# Autodesk Inventor assembly: prowadzenie
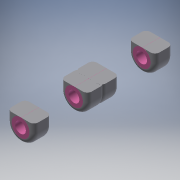
[picture p0: Inventor's stored thumbnail of the model, 180x180]
Saved by Autodesk Inventor 2019 (Build 230136000, 136)
## iProperties
Created: 2020-01-12
Part Number: prowadzenie
Material: Ogólny
Document SubType Name: Assembly
Designer: Karolina
Author: Karolina
## Documents named in this file (3)
- C:\Users\Karolina\Desktop\Kuba\rekav2\dlon\prowadzenie.iam
- C:\Users\Karolina\Desktop\Kuba\rekav2\dlon\lozysko.ipt
- C:\Users\Karolina\Desktop\Kuba\rekav2\dlon\trzym.ipt
## Components (8 placed, 2 different names)
1. trzym:1 — Równoległy:3, Zestawiający:3, Zestawiający:5, Zestawiający:8, Równoległy:5
2. trzym:2 — Równoległy:2, Zestawiający:3, Zestawiający:4, Zestawiający:6, Zestawiający:7, Równoległy:7
3. trzym:3 — Zestawiający:1, Zestawiający:2, Równoległy:1, Równoległy:2, Zestawiający:6, Zestawiający:9, Zestawiający:10, Równoległy:4
4. trzym:4 — Zestawiający:1, Zestawiający:2, Równoległy:1, Równoległy:3, Zestawiający:4, Zestawiający:5, Równoległy:6
5. lozysko:1 — Zestawiający:10, Równoległy:4
6. lozysko:2 — Zestawiający:9, Równoległy:6
7. lozysko:3 — Zestawiający:8, Równoległy:7
8. lozysko:4 — Zestawiający:7, Równoległy:5
## Relationships (17: Mate 10, Flush 7)
- Zestawiający:1 [Mate] (-0.2 mm): trzym:3 ↔ trzym:4
- Zestawiający:2 [Mate]: trzym:3 ↔ trzym:4
- Równoległy:1 [Flush]: trzym:3 ↔ trzym:4
- Równoległy:2 [Flush]: trzym:2 ↔ trzym:3
- Równoległy:3 [Flush]: trzym:1 ↔ trzym:4
- Zestawiający:3 [Mate]: trzym:1 ↔ trzym:2
- Zestawiający:4 [Mate]: trzym:2 ↔ trzym:4
- Zestawiający:5 [Mate] (2 mm): trzym:1 ↔ trzym:4
- Zestawiający:6 [Mate] (2 mm): trzym:2 ↔ trzym:3
- Zestawiający:7 [Mate]: trzym:2 ↔ lozysko:4
- Zestawiający:8 [Mate]: trzym:1 ↔ lozysko:3
- Zestawiający:9 [Mate]: trzym:3 ↔ lozysko:2
- Zestawiający:10 [Mate]: trzym:3 ↔ lozysko:1
- Równoległy:4 [Flush]: trzym:3 ↔ lozysko:1
- Równoległy:5 [Flush]: trzym:1 ↔ lozysko:4
- Równoległy:6 [Flush]: trzym:4 ↔ lozysko:2
- Równoległy:7 [Flush]: trzym:2 ↔ lozysko:3
